# Autodesk Inventor assembly: Head
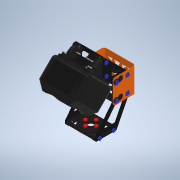
[picture p0: Inventor's stored thumbnail of the model, 180x180]
Saved by Autodesk Inventor 2020.4 (Build 244396000, 396)
## iProperties
Created: 2021-12-31
Part Number: Head
Document SubType Name: Assembly
Designer: Masato Kubotera
Mass: 92.9564 g
Surface Area: 535.434 cm^2
Volume: 94.1049 cm^3
Density: 0.987795 g/cm^3
Author: Masato Kubotera
## Documents named in this file (17)
- C:\Users\Masato\Desktop\SUSTAINA-OP\UpperBody\Head\Head.iam
- C:\Users\Masato\Desktop\SUSTAINA-OP\UpperBody\Head\CameraUnit_e-CAM50_CUNX.iam
- C:\Users\Masato\Desktop\SUSTAINA-OP\UpperBody\Head\Camera_side_frame.ipt
- C:\Users\Masato\Desktop\SUSTAINA-OP\ReadyMade\InsertNut\UD-43040.ipt
- C:\Users\Masato\Desktop\SUSTAINA-OP\UpperBody\Head\Head_side_frame.ipt
- C:\Users\Masato\Desktop\SUSTAINA-OP\ReadyMade\Screw\M3-6.ipt
- C:\Users\Masato\Desktop\SUSTAINA-OP\UpperBody\Head\Head_horn_frame.ipt
- C:\Users\Masato\Desktop\SUSTAINA-OP\ReadyMade\InsertNut\IRU-304S.ipt
- C:\Users\Masato\Desktop\SUSTAINA-OP\ReadyMade\Washer\TT-2532-10.ipt
- C:\Users\Masato\Desktop\SUSTAINA-OP\ReadyMade\Screw\M2_6-8.ipt
- C:\Users\Masato\Desktop\SUSTAINA-OP\UpperBody\Head\Head_diagonal.ipt
- C:\Users\Masato\Desktop\SUSTAINA-OP\UpperBody\Head\Fan_support_stand.ipt
- C:\Users\Masato\Desktop\SUSTAINA-OP\ReadyMade\YDM2507C12F.ipt
- C:\Users\Masato\Desktop\SUSTAINA-OP\ReadyMade\Screw\M3-10.ipt
- C:\Users\Masato\Desktop\SUSTAINA-OP\ReadyMade\Bush\L3040-8110TB.ipt
- C:\Users\Masato\Desktop\SUSTAINA-OP\ReadyMade\Screw\M3-8.ipt
- C:\Users\Masato\Desktop\SUSTAINA-OP\UpperBody\Head\Head_GK_cloth.ipt
## Components (60 placed, 16 different names)
1. CameraUnit_e-CAM50_CUNX:1 [sub-assembly] — 挿入:1, 挿入:2, 挿入:3, 挿入:4
2. Camera_side_frame:1 — 挿入:1, 挿入:2, 挿入:5, 挿入:6, 挿入:62, 挿入:64
3. Camera_side_frame:2 — 挿入:3, 挿入:4, 挿入:7, 挿入:8, 挿入:63, 挿入:65
4. Head_side_frame:1 — 挿入:13, 挿入:14, 挿入:17, 挿入:18, 挿入:25, 挿入:26, 挿入:34, 挿入:35, 挿入:46, 挿入:47, 挿入:52, 挿入:53, 挿入:54, 挿入:58, 挿入:78, 挿入:79
5. Head_side_frame:2 — 挿入:15, 挿入:16, 挿入:19, 挿入:20, 挿入:27, 挿入:28, 挿入:36, 挿入:37, 挿入:48, 挿入:49, 挿入:50, 挿入:51, 挿入:56, 挿入:60, 挿入:80, 挿入:81
6. Head_diagonal:1 — 挿入:38, 挿入:39, 挿入:40, 挿入:41
7. Head_diagonal:2 — 挿入:42, 挿入:43, 挿入:44, 挿入:45
8. Head_horn_frame:1 — 挿入:21, 挿入:22, 挿入:23, 挿入:24, 挿入:29, 挿入:30, 挿入:31, 挿入:32, 挿入:33, メイト:1, メイト:2, メイト:3
9. TT-2532-10:1 — 挿入:29
10. Fan_support_stand:1 — 挿入:62, 挿入:63, 挿入:64, 挿入:65, 挿入:66, 挿入:67, 挿入:68, 挿入:69, 挿入:70, 挿入:71, 挿入:72, 挿入:73
11. YDM2507C12F:1 — 挿入:66, 挿入:67, 挿入:68, 挿入:69, 挿入:74, 挿入:75, 挿入:76, 挿入:77
12. M3-10:1 — 挿入:70
13. M3-10:2 — 挿入:71
14. M3-10:3 — 挿入:72
15. M3-10:4 — 挿入:73
16. M3-10:5 — 挿入:74
17. M3-10:6 — 挿入:75
18. M3-10:7 — 挿入:76
19. M3-10:8 — 挿入:77
20. L3040-8110TB:1 — 挿入:78, 挿入:82, 挿入:86
21. L3040-8110TB:2 — 挿入:79, 挿入:83, 挿入:87
22. L3040-8110TB:3 — 挿入:80, 挿入:84
23. L3040-8110TB:4 — 挿入:81, 挿入:85
24. M3-8:1 — 挿入:83
25. M3-8:2 — 挿入:82
26. M3-8:3 — 挿入:84
27. M3-8:4 — 挿入:85
28. Head_GK_cloth:1 — 挿入:86, 挿入:87
29. M3-6:1 — 挿入:17
30. M3-6:2 — 挿入:18
31. M3-6:3 — 挿入:19
32. M3-6:4 — 挿入:20
33. M3-6:5 — 挿入:34
34. M3-6:6 — 挿入:35
35. M3-6:7 — 挿入:36
36. M3-6:8 — 挿入:37
37. M3-6:9 — 挿入:54
38. M3-6:11 — 挿入:56
39. M3-6:13 — 挿入:58
40. M3-6:15 — 挿入:60
41. M2_6-8:1 — 挿入:30
42. M2_6-8:2 — 挿入:31
43. M2_6-8:3 — 挿入:32
44. M2_6-8:4 — 挿入:33
45. UD-43040:1 — 挿入:5, 挿入:13
46. UD-43040:2 — 挿入:6, 挿入:14
47. UD-43040:3 — 挿入:7, 挿入:15
48. UD-43040:4 — 挿入:8, 挿入:16
49. IRU-304S:1 — 挿入:21, 挿入:25
50. IRU-304S:2 — 挿入:22, 挿入:26
51. IRU-304S:3 — 挿入:23, 挿入:28
52. IRU-304S:4 — 挿入:24, 挿入:27
53. IRU-304S:5 — 挿入:38, 挿入:46
54. IRU-304S:6 — 挿入:39, 挿入:47
55. IRU-304S:7 — 挿入:40, 挿入:48
56. IRU-304S:8 — 挿入:41, 挿入:49
57. IRU-304S:9 — 挿入:42, 挿入:53
58. IRU-304S:10 — 挿入:43, 挿入:52
59. IRU-304S:11 — 挿入:44, 挿入:50
60. IRU-304S:12 — 挿入:45, 挿入:51
## Relationships (82: Insert 79, Mate 3)
- 挿入:1 [Insert]: CameraUnit_e-CAM50_CUNX:1 ↔ Camera_side_frame:1
- 挿入:2 [Insert]: CameraUnit_e-CAM50_CUNX:1 ↔ Camera_side_frame:1
- 挿入:3 [Insert]: CameraUnit_e-CAM50_CUNX:1 ↔ Camera_side_frame:2
- 挿入:4 [Insert]: CameraUnit_e-CAM50_CUNX:1 ↔ Camera_side_frame:2
- 挿入:5 [Insert]: Camera_side_frame:1 ↔ UD-43040:1
- 挿入:6 [Insert]: Camera_side_frame:1 ↔ UD-43040:2
- 挿入:7 [Insert]: Camera_side_frame:2 ↔ UD-43040:3
- 挿入:8 [Insert]: Camera_side_frame:2 ↔ UD-43040:4
- 挿入:13 [Insert]: Head_side_frame:1 ↔ UD-43040:1
- 挿入:14 [Insert]: Head_side_frame:1 ↔ UD-43040:2
- 挿入:15 [Insert]: Head_side_frame:2 ↔ UD-43040:3
- 挿入:16 [Insert]: Head_side_frame:2 ↔ UD-43040:4
- 挿入:17 [Insert]: Head_side_frame:1 ↔ M3-6:1
- 挿入:18 [Insert]: Head_side_frame:1 ↔ M3-6:2
- 挿入:19 [Insert]: Head_side_frame:2 ↔ M3-6:3
- 挿入:20 [Insert]: Head_side_frame:2 ↔ M3-6:4
- 挿入:21 [Insert]: Head_horn_frame:1 ↔ IRU-304S:1
- 挿入:22 [Insert]: Head_horn_frame:1 ↔ IRU-304S:2
- 挿入:23 [Insert]: Head_horn_frame:1 ↔ IRU-304S:3
- 挿入:24 [Insert]: Head_horn_frame:1 ↔ IRU-304S:4
- 挿入:25 [Insert]: Head_side_frame:1 ↔ IRU-304S:1
- 挿入:26 [Insert]: Head_side_frame:1 ↔ IRU-304S:2
- 挿入:27 [Insert]: Head_side_frame:2 ↔ IRU-304S:4
- 挿入:28 [Insert]: Head_side_frame:2 ↔ IRU-304S:3
- 挿入:29 [Insert]: Head_horn_frame:1 ↔ TT-2532-10:1
- 挿入:30 [Insert]: Head_horn_frame:1 ↔ M2_6-8:1
- 挿入:31 [Insert]: Head_horn_frame:1 ↔ M2_6-8:2
- 挿入:32 [Insert]: Head_horn_frame:1 ↔ M2_6-8:3
- 挿入:33 [Insert]: Head_horn_frame:1 ↔ M2_6-8:4
- 挿入:34 [Insert]: Head_side_frame:1 ↔ M3-6:5
- 挿入:35 [Insert]: Head_side_frame:1 ↔ M3-6:6
- 挿入:36 [Insert]: Head_side_frame:2 ↔ M3-6:7
- 挿入:37 [Insert]: Head_side_frame:2 ↔ M3-6:8
- 挿入:38 [Insert]: Head_diagonal:1 ↔ IRU-304S:5
- 挿入:39 [Insert]: Head_diagonal:1 ↔ IRU-304S:6
- 挿入:40 [Insert]: Head_diagonal:1 ↔ IRU-304S:7
- 挿入:41 [Insert]: Head_diagonal:1 ↔ IRU-304S:8
- 挿入:42 [Insert]: Head_diagonal:2 ↔ IRU-304S:9
- 挿入:43 [Insert]: Head_diagonal:2 ↔ IRU-304S:10
- 挿入:44 [Insert]: Head_diagonal:2 ↔ IRU-304S:11
- 挿入:45 [Insert]: Head_diagonal:2 ↔ IRU-304S:12
- 挿入:46 [Insert]: Head_side_frame:1 ↔ IRU-304S:5
- 挿入:47 [Insert]: Head_side_frame:1 ↔ IRU-304S:6
- 挿入:48 [Insert]: Head_side_frame:2 ↔ IRU-304S:7
- 挿入:49 [Insert]: Head_side_frame:2 ↔ IRU-304S:8
- 挿入:50 [Insert]: Head_side_frame:2 ↔ IRU-304S:11
- 挿入:51 [Insert]: Head_side_frame:2 ↔ IRU-304S:12
- 挿入:52 [Insert]: Head_side_frame:1 ↔ IRU-304S:10
- 挿入:53 [Insert]: Head_side_frame:1 ↔ IRU-304S:9
- 挿入:54 [Insert]: Head_side_frame:1 ↔ M3-6:9
- 挿入:56 [Insert]: Head_side_frame:2 ↔ M3-6:11
- 挿入:58 [Insert]: Head_side_frame:1 ↔ M3-6:13
- 挿入:60 [Insert]: Head_side_frame:2 ↔ M3-6:15
- メイト:1 [Mate]: Head_horn_frame:1
- メイト:2 [Mate]: Head_horn_frame:1
- メイト:3 [Mate]: Head_horn_frame:1
- 挿入:62 [Insert]: Camera_side_frame:1 ↔ Fan_support_stand:1
- 挿入:63 [Insert]: Camera_side_frame:2 ↔ Fan_support_stand:1
- 挿入:64 [Insert]: Camera_side_frame:1 ↔ Fan_support_stand:1
- 挿入:65 [Insert]: Camera_side_frame:2 ↔ Fan_support_stand:1
- 挿入:66 [Insert]: Fan_support_stand:1 ↔ YDM2507C12F:1
- 挿入:67 [Insert]: Fan_support_stand:1 ↔ YDM2507C12F:1
- 挿入:68 [Insert]: Fan_support_stand:1 ↔ YDM2507C12F:1
- 挿入:69 [Insert]: Fan_support_stand:1 ↔ YDM2507C12F:1
- 挿入:70 [Insert]: Fan_support_stand:1 ↔ M3-10:1
- 挿入:71 [Insert]: Fan_support_stand:1 ↔ M3-10:2
- 挿入:72 [Insert]: Fan_support_stand:1 ↔ M3-10:3
- 挿入:73 [Insert]: Fan_support_stand:1 ↔ M3-10:4
- 挿入:74 [Insert]: YDM2507C12F:1 ↔ M3-10:5
- 挿入:75 [Insert]: YDM2507C12F:1 ↔ M3-10:6
- 挿入:76 [Insert]: YDM2507C12F:1 ↔ M3-10:7
- 挿入:77 [Insert]: YDM2507C12F:1 ↔ M3-10:8
- 挿入:78 [Insert]: Head_side_frame:1 ↔ L3040-8110TB:1
- 挿入:79 [Insert]: Head_side_frame:1 ↔ L3040-8110TB:2
- 挿入:80 [Insert]: Head_side_frame:2 ↔ L3040-8110TB:3
- 挿入:81 [Insert]: Head_side_frame:2 ↔ L3040-8110TB:4
- 挿入:82 [Insert]: L3040-8110TB:1 ↔ M3-8:2
- 挿入:83 [Insert]: L3040-8110TB:2 ↔ M3-8:1
- 挿入:84 [Insert]: L3040-8110TB:3 ↔ M3-8:3
- 挿入:85 [Insert]: L3040-8110TB:4 ↔ M3-8:4
- 挿入:86 [Insert]: L3040-8110TB:1 ↔ Head_GK_cloth:1
- 挿入:87 [Insert]: L3040-8110TB:2 ↔ Head_GK_cloth:1
